# Autodesk Inventor assembly: ZDrive
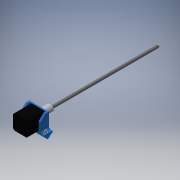
[picture p0: Inventor's stored thumbnail of the model, 180x180]
Saved by Autodesk Inventor 2016 (Build 200138000, 138)
## iProperties
Created: 2015-01-30
Part Number: ZDrive
Document SubType Name: Assembly
Designer: Jack
Mass: 256.814 g
Surface Area: 386.968 cm^2
Volume: 133.337 cm^3
Density: 1.92604 g/cm^3
Author: Jack
Title: Z Drive
## Documents named in this file (7)
- C:\Users\Jack\ownCloud\Projects\CrossBot\InventorModel\ZAxis\ZDrive.iam
- C:\Users\Jack\ownCloud\Projects\CrossBot\InventorModel\Electronics\Motors\StepperMotorNema17x48mm.ipt
- C:\Users\Jack\ownCloud\Projects\CrossBot\InventorModel\Hardware\ZDrive\ZACMEScrew.ipt
- C:\Users\Jack\ownCloud\Projects\CrossBot\InventorModel\ZAxis\ZMotorMount.ipt
- C:\Users\Jack\ownCloud\Projects\CrossBot\InventorModel\Hardware\BoltWashers\BoltWasher4\BoltWasher4x10.iam
- C:\Users\Jack\ownCloud\Projects\CrossBot\InventorModel\Hardware\BoltWashers\BoltWasher3\BoltWasher3x8.iam
- C:\Users\Jack\ownCloud\Projects\CrossBot\InventorModel\Hardware\ZDrive\ZACMEFlexCoupler.ipt
## Components (12 placed, 6 different names)
1. StepperMotorNema17x48mm:1 — Mate:6, Mate:7, Mate:8, Mate:9, Mate:27, Mate:28, Mate:30
2. ZACMEScrew:1 — Mate:27, Mate:29, Mate:30
3. ZMotorMount:1 — Mate:6, Mate:7, Mate:8, Mate:9, Mate:10, Mate:11, Mate:12, Mate:13, Mate:14, Mate:15, Mate:16, Mate:17, Mate:18, Mate:19, Mate:20, Mate:21, Mate:22, Mate:23, Mate:24, Mate:25
4. ZACMEFlexCoupler:1 — Mate:28, Mate:29
5. BoltWasher3x8:1 [sub-assembly] — Mate:19, Mate:25
6. BoltWasher3x8:2 [sub-assembly] — Mate:21, Mate:23
7. BoltWasher3x8:3 [sub-assembly] — Mate:18, Mate:24
8. BoltWasher3x8:4 [sub-assembly] — Mate:20, Mate:22
9. BoltWasher4x10:1 [sub-assembly] — Mate:12, Mate:17
10. BoltWasher4x10:2 [sub-assembly] — Mate:13, Mate:14
11. BoltWasher4x10:4 [sub-assembly] — Mate:11, Mate:16
12. BoltWasher4x10:3 [sub-assembly] — Mate:10, Mate:15
## Relationships (25: Mate 25)
- [Mate]: StepperMotorNema17x48mm:1 ↔ ZMotorMount:1
- Mate:6: StepperMotorNema17x48mm:1 ↔ ZMotorMount:1
- Mate:7: StepperMotorNema17x48mm:1 ↔ ZMotorMount:1
- Mate:8: StepperMotorNema17x48mm:1 ↔ ZMotorMount:1
- Mate:9: StepperMotorNema17x48mm:1 ↔ ZMotorMount:1
- Mate:10: ZMotorMount:1 ↔ BoltWasher4x10:3
- Mate:11: ZMotorMount:1 ↔ BoltWasher4x10:4
- Mate:12: ZMotorMount:1 ↔ BoltWasher4x10:1
- Mate:13: ZMotorMount:1 ↔ BoltWasher4x10:2
- Mate:14: ZMotorMount:1 ↔ BoltWasher4x10:2
- Mate:15: ZMotorMount:1 ↔ BoltWasher4x10:3
- Mate:16: ZMotorMount:1 ↔ BoltWasher4x10:4
- Mate:17: ZMotorMount:1 ↔ BoltWasher4x10:1
- Mate:18: ZMotorMount:1 ↔ BoltWasher3x8:3
- Mate:19: ZMotorMount:1 ↔ BoltWasher3x8:1
- Mate:20: ZMotorMount:1 ↔ BoltWasher3x8:4
- Mate:21: ZMotorMount:1 ↔ BoltWasher3x8:2
- Mate:22: ZMotorMount:1 ↔ BoltWasher3x8:4
- Mate:23: ZMotorMount:1 ↔ BoltWasher3x8:2
- Mate:24: ZMotorMount:1 ↔ BoltWasher3x8:3
- Mate:25: ZMotorMount:1 ↔ BoltWasher3x8:1
- Mate:27: StepperMotorNema17x48mm:1 ↔ ZACMEScrew:1
- Mate:28: StepperMotorNema17x48mm:1 ↔ ZACMEFlexCoupler:1
- Mate:29: ZACMEScrew:1 ↔ ZACMEFlexCoupler:1
- Mate:30: StepperMotorNema17x48mm:1 ↔ ZACMEScrew:1
